# Autodesk Inventor assembly: CIM Motor 14T
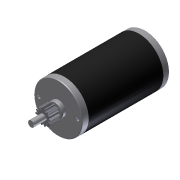
[picture p0: Inventor's stored thumbnail of the model, 180x180]
Saved by Autodesk Inventor 2011 (Build 150239000, 239)
## iProperties
Created: 2012-05-20
Part Number: CIM Motor 14T
Document SubType Name: Assembly
Designer: Nemo
Author: Nemo
## Documents named in this file (3)
- H:\Nemo\Documents\Robotics\COTS Parts\Motors\CIM Motor 14T.iam
- H:\Nemo\Documents\Robotics\Motors\CIM motor.ipt
- H:\Nemo\Documents\Robotics\COTS Parts\Gearboxes\Gears\Gear 20dp 8mm key 14T.ipt
## Components (2 placed, 2 different names)
1. CIM motor:1 — Mate:1, Flush:1, Mate:2
2. 14T CIM Gear — Mate:1, Flush:1, Mate:2
## Relationships (3: Mate 2, Flush 1)
- Mate:1: CIM motor:1 ↔ 14T CIM Gear
- Flush:1: CIM motor:1 ↔ 14T CIM Gear
- Mate:2 (3.175 mm): CIM motor:1 ↔ 14T CIM Gear
